# Autodesk Inventor assembly: airhockeybot_x_traverse_sumulation
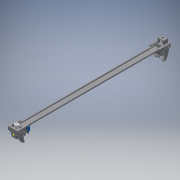
[picture p0: Inventor's stored thumbnail of the model, 180x180]
Saved by Autodesk Inventor 2019.3 (Build 233278000, 278)
## iProperties
Created: 2020-08-23
Part Number: airhockeybot_x_traverse_sumulation
Material: Generisch
Document SubType Name: Assembly
Designer: Nicolas Frick
Author: Nicolas Frick
## Documents named in this file (14)
- C:\Users\Nicolas Frick\Sync\OneDrive\airhockeybot\mechanical_design\common_cad_parts\sim_models\airhockeybot_x_traverse_sumulation.iam
- C:\Users\Nicolas Frick\Sync\OneDrive\airhockeybot\mechanical_design\inventor\Pulley.iam
- C:\Users\Nicolas Frick\Sync\OneDrive\airhockeybot\mechanical_design\inventor\Switch CMV101D\CNDT_CMV101D.ipt
- C:\Users\Nicolas Frick\Sync\OneDrive\airhockeybot\mechanical_design\inventor\Nema 17HS5425\Assembly1.iam
- C:\Users\Nicolas Frick\Sync\OneDrive\airhockeybot\mechanical_design\inventor\GT2 40T 5mm Bore 6mm wide pulley\GT2 40T 5 Bore v2.iam
- C:\Users\Nicolas Frick\Sync\OneDrive\airhockeybot\mechanical_design\inventor\igus\WS_10_40_200_2_modify.ipt
- C:\Users\Nicolas Frick\Sync\OneDrive\airhockeybot\mechanical_design\inventor\Upper_left_fixture.ipt
- C:\Users\Nicolas Frick\Sync\OneDrive\airhockeybot\mechanical_design\inventor\Belt_clamp.ipt
- C:\Users\Nicolas Frick\Sync\OneDrive\airhockeybot\mechanical_design\inventor\Belt_clamp_mirrored.ipt
- C:\Users\Nicolas Frick\Sync\OneDrive\airhockeybot\mechanical_design\inventor\Upper_right_fixture.ipt
- C:\Users\Nicolas Frick\Sync\OneDrive\airhockeybot\mechanical_design\inventor\Upper_bearing_support_inside.ipt
- C:\Users\Nicolas Frick\Sync\OneDrive\airhockeybot\mechanical_design\inventor\Upper_bearing_support_outside.ipt
- C:\Users\Nicolas Frick\Sync\OneDrive\airhockeybot\mechanical_design\inventor\Stiff_motor.ipt
- C:\Users\Nicolas Frick\Sync\OneDrive\airhockeybot\mechanical_design\inventor\Stiff.ipt
## Components (15 placed, 13 different names)
1. WS_10_40_200_2_modify:1 — Passend:187, Passend:188, Passend:189
2. Upper_left_fixture:1 — Fluchtend:38, Fluchtend:39, Fluchtend:40, Fluchtend:44, Passend:146, Passend:147, Passend:187, Passend:189, Passend:191, Fluchtend:75, Fluchtend:76
3. Assembly1:3 [sub-assembly] — Passend:105, Passend:106, Fluchtend:38, Fluchtend:39, Fluchtend:40
4. GT2 40T 5 Bore v2:3 [sub-assembly] — Passend:105, Passend:106
5. Belt_clamp:1 — Fluchtend:41, Fluchtend:42, Passend:147, Passend:195, Passend:197, Passend:198
6. Belt_clamp_mirrored:1 — Fluchtend:41, Fluchtend:42, Passend:146
7. Upper_right_fixture:1 — Fluchtend:44, Passend:131, Passend:132, Passend:144, Passend:145, Passend:188
8. Upper_bearing_support_inside:1 — Passend:127, Passend:128, Fluchtend:48, Fluchtend:49, Passend:130, Passend:131, Passend:132
9. Pulley:3 [sub-assembly] — Passend:127, Passend:128, Passend:129
10. Upper_bearing_support_outside:1 — Fluchtend:48, Fluchtend:49, Passend:129, Passend:130
11. Belt_clamp:2 — Fluchtend:50, Fluchtend:51, Passend:144, Passend:206, Passend:208
12. Belt_clamp_mirrored:2 — Fluchtend:50, Fluchtend:51, Passend:145, Passend:207
13. CNDT_CMV101D:6 — Passend:191, Fluchtend:75, Fluchtend:76
14. Stiff_motor:1 — Passend:195, Passend:197, Passend:198
15. Stiff:1 — Passend:206, Passend:207, Passend:208
## Relationships (34: Mate 22, Flush 12)
- Passend:105 [Mate]: Assembly1:3 ↔ GT2 40T 5 Bore v2:3
- Passend:106 [Mate] (1.3 mm): Assembly1:3 ↔ GT2 40T 5 Bore v2:3
- Fluchtend:38 [Flush] (13 mm): Upper_left_fixture:1 ↔ Assembly1:3
- Fluchtend:39 [Flush] (5 mm): Upper_left_fixture:1 ↔ Assembly1:3
- Fluchtend:40 [Flush] (10 mm): Upper_left_fixture:1 ↔ Assembly1:3
- Fluchtend:41 [Flush]: Belt_clamp:1 ↔ Belt_clamp_mirrored:1
- Fluchtend:42 [Flush]: Belt_clamp:1 ↔ Belt_clamp_mirrored:1
- Fluchtend:44 [Flush]: Upper_left_fixture:1 ↔ Upper_right_fixture:1
- Passend:127 [Mate]: Upper_bearing_support_inside:1 ↔ Pulley:3
- Passend:128 [Mate]: Upper_bearing_support_inside:1 ↔ Pulley:3
- Fluchtend:48 [Flush]: Upper_bearing_support_inside:1 ↔ Upper_bearing_support_outside:1
- Fluchtend:49 [Flush]: Upper_bearing_support_inside:1 ↔ Upper_bearing_support_outside:1
- Passend:129 [Mate]: Pulley:3 ↔ Upper_bearing_support_outside:1
- Passend:130 [Mate]: Upper_bearing_support_inside:1 ↔ Upper_bearing_support_outside:1
- Passend:131 [Mate] (0.1 mm): Upper_right_fixture:1 ↔ Upper_bearing_support_inside:1
- Passend:132 [Mate]: Upper_right_fixture:1 ↔ Upper_bearing_support_inside:1
- Fluchtend:50 [Flush]: Belt_clamp:2 ↔ Belt_clamp_mirrored:2
- Fluchtend:51 [Flush]: Belt_clamp:2 ↔ Belt_clamp_mirrored:2
- Passend:144 [Mate]: Upper_right_fixture:1 ↔ Belt_clamp:2
- Passend:145 [Mate]: Upper_right_fixture:1 ↔ Belt_clamp_mirrored:2
- Passend:146 [Mate]: Upper_left_fixture:1 ↔ Belt_clamp_mirrored:1
- Passend:147 [Mate]: Upper_left_fixture:1 ↔ Belt_clamp:1
- Passend:187 [Mate]: WS_10_40_200_2_modify:1 ↔ Upper_left_fixture:1
- Passend:188 [Mate]: WS_10_40_200_2_modify:1 ↔ Upper_right_fixture:1
- Passend:189 [Mate]: WS_10_40_200_2_modify:1 ↔ Upper_left_fixture:1
- Passend:191 [Mate]: Upper_left_fixture:1 ↔ CNDT_CMV101D:6
- Fluchtend:75 [Flush] (1 mm): Upper_left_fixture:1 ↔ CNDT_CMV101D:6
- Fluchtend:76 [Flush] (4 mm): Upper_left_fixture:1 ↔ CNDT_CMV101D:6
- Passend:195 [Mate]: Belt_clamp:1 ↔ Stiff_motor:1
- Passend:197 [Mate]: Belt_clamp:1 ↔ Stiff_motor:1
- Passend:198 [Mate]: Belt_clamp:1 ↔ Stiff_motor:1
- Passend:206 [Mate]: Belt_clamp:2 ↔ Stiff:1
- Passend:207 [Mate]: Belt_clamp_mirrored:2 ↔ Stiff:1
- Passend:208 [Mate]: Belt_clamp:2 ↔ Stiff:1
